# Autodesk Inventor assembly: 10-SUSP-04_MIR_MIR
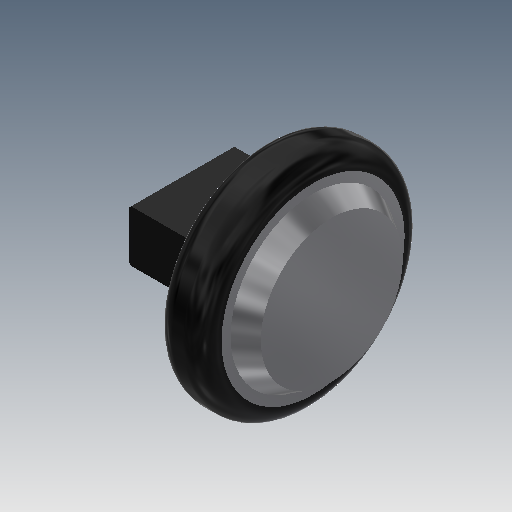
[picture p0: Inventor's stored thumbnail of the model, 512x512]
Saved by Autodesk Inventor 2018 (Build 220112000, 112)
## iProperties
Created: 2017-07-31
Part Number: 10-SUSP-04_MIR_MIR
Document SubType Name: Assembly
Designer: feesmrt
Author: feesmrt
## Documents named in this file (3)
- C:\Users\feesmrt\Documents\NRBDL\Inventor-NRBDL\10-SUSP\10-SUSP-04_MIR_MIR.iam
- C:\Users\feesmrt\Documents\NRBDL\Inventor-NRBDL\10-SUSP\10-006-ACTR-FIX_MIR.ipt
- C:\Users\feesmrt\Documents\NRBDL\Inventor-NRBDL\10-SUSP\10-001-ACTR_MIR.ipt
## Components (2 placed, 2 different names)
1. 10-006-ACTR-FIX_MIR:1 — Mate:2, Angle:2, Angle:1, Mate:1
2. 10-001-ACTR_MIR:1 — Mate:2, Angle:2, Angle:1, Mate:1
## Relationships (4: Mate 2, Angle 2)
- Mate:2: 10-006-ACTR-FIX_MIR:1 ↔ 10-001-ACTR_MIR:1
- Angle:2 (0 deg): 10-006-ACTR-FIX_MIR:1 ↔ 10-001-ACTR_MIR:1
- Angle:1 (0 deg): 10-006-ACTR-FIX_MIR:1 ↔ 10-001-ACTR_MIR:1
- Mate:1: 10-006-ACTR-FIX_MIR:1 ↔ 10-001-ACTR_MIR:1
